# Autodesk Inventor assembly: 25-Armor
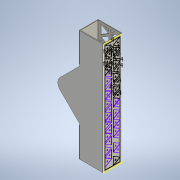
[picture p0: Inventor's stored thumbnail of the model, 180x180]
Saved by Autodesk Inventor 2022 (Build 260153000, 153)
## iProperties
Created: 2022-08-14
Part Number: 25-Armor
Document SubType Name: Assembly
Designer: Nick
Mass: 518.131 g
Surface Area: 1219.97 cm^2
Volume: 105.569 cm^3
Density: 4.90796 g/cm^3
Author: Nick
## Documents named in this file (3)
- Y:\Projects\BattleBot\25-Armor.iam
- Y:\Projects\BattleBot\Top Armor.ipt
- Y:\Projects\BattleBot\Base Plate.ipt
## Components (2 placed, 2 different names)
1. Top Armor:1 — Flush:1, Flush:2, Mate:1
2. Base Plate:1 — Flush:1, Flush:2, Mate:1
## Relationships (3: Flush 2, Mate 1)
- Flush:1: Top Armor:1 ↔ Base Plate:1
- Flush:2: Top Armor:1 ↔ Base Plate:1
- Mate:1: Top Armor:1 ↔ Base Plate:1
